# Autodesk Inventor assembly: Outer
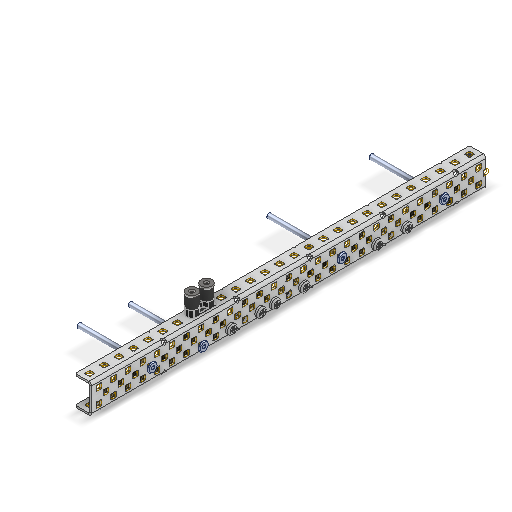
[picture p0: Inventor's stored thumbnail of the model, 512x512]
Saved by Autodesk Inventor 2025.2 (Build 292293000, 293)
## iProperties
Created: 2025-01-27
Part Number: Outer
Document SubType Name: Assembly
Designer: Averey Ku
Author: Averey Ku
## Documents named in this file (19)
- C:\Users\avere\VEX-CAD\V5-CAD\V0.2\Drivetrain\Drivebay Left\Outer.iam
- C:\Users\avere\VEX-CAD\ROBOPROS-CAD-Inventor\Motion\Shaft LS\Bearing Flat Low Profile.ipt
- C:\Users\avere\VEX-CAD\ROBOPROS-CAD-Inventor\Structure\Hardware\Screw Nylon - Pan Head\NScrew Pan Head Threaded .500.ipt
- C:\Users\avere\VEX-CAD\ROBOPROS-CAD-Inventor\Structure\Hardware\Screw Steel - Star\SScrew Star Smooth 2.500.ipt
- C:\Users\avere\VEX-CAD\ROBOPROS-CAD-Inventor\Structure\Hardware\Nut Keps.ipt
- C:\Users\avere\VEX-CAD\ROBOPROS-CAD-Inventor\Structure\Hardware\Nut Nylon\Nut Nylon - White.ipt
- C:\Users\avere\VEX-CAD\ROBOPROS-CAD-Inventor\Structure\C Channel\Aluminum 1x2x1\Alu C 1x2x1x28.ipt
- C:\Users\avere\VEX-CAD\ROBOPROS-CAD-Inventor\Structure\Standoff\Standoff .875.ipt
- C:\Users\avere\VEX-CAD\ROBOPROS-CAD-Inventor\Modified Parts\Bearing Flat Low Profile 2-Hole.ipt
- C:\Users\avere\VEX-CAD\ROBOPROS-CAD-Inventor\Motion\Spacers\Spacer Nylon .375 OD\NSpacer .375 OD x .375.ipt
- C:\Users\avere\VEX-CAD\ROBOPROS-CAD-Inventor\Motion\Spacers\Washer Steel\SWasher .375 OD x .062500.ipt
- C:\Users\avere\VEX-CAD\ROBOPROS-CAD-Inventor\Structure\Hardware\Screw Alu - Slotted\AScrew Slotted Threaded .250.ipt
- C:\Users\avere\VEX-CAD\ROBOPROS-CAD-Inventor\Structure\C Channel\Aluminum 1x2x1\Alu C 1x2x1x27.ipt
- C:\Users\avere\VEX-CAD\ROBOPROS-CAD-Inventor\Structure\Nylon Standoff Rounded\Nylon Standoff .875.ipt
- C:\Users\avere\VEX-CAD\ROBOPROS-CAD-Inventor\Structure\Hardware\Screw Steel - Star.ipt
- C:\Users\avere\VEX-CAD\ROBOPROS-CAD-Inventor\Structure\Hardware\Nut Nylon.ipt
- C:\Users\avere\VEX-CAD\ROBOPROS-CAD-Inventor\Structure\Standoff.ipt
- C:\Users\avere\VEX-CAD\ROBOPROS-CAD-Inventor\Motion\Spacers\Spacer Nylon .375 OD.ipt
- C:\Users\avere\VEX-CAD\ROBOPROS-CAD-Inventor\Motion\Spacers\Washer Steel.ipt
## Components (32 placed, 13 different names)
1. Bearing Flat Low Profile:2 — Insert:21, Insert:22, Insert:32, Mate:3
2. Bearing Flat Low Profile:3 — Insert:23, Insert:24, Insert:44
3. NScrew Pan Head Threaded .500:2 — Insert:35
4. NScrew Pan Head Threaded .500:3 — Insert:37
5. NScrew Pan Head Threaded .500:4 — Insert:36
6. NScrew Pan Head Threaded .500:5 — Insert:39, Mate:4
7. NScrew Pan Head Threaded .500:6 — Insert:38
8. SScrew Star Smooth 2.500:1 — Insert:27
9. SScrew Star Smooth 2.500:3 — Insert:26
10. SScrew Star Smooth 2.500:4 — Insert:25
11. Nut Keps:2 — Insert:43
12. Nut Keps:3 — Insert:41
13. Nut Keps:4 — Insert:42
14. Nut Nylon - White:2 — Insert:21
15. Nut Nylon - White:4 — Insert:22
16. Nut Nylon - White:5 — Insert:23, Mate:4
17. Nut Nylon - White:6 — Insert:24
18. Alu C 1x2x1x28:1 — Flush:1, Flush:2, Flush:3, Insert:25, Insert:26, Insert:27, Insert:31, Mate:2, Insert:32, Mate:3, Insert:35, Insert:36, Insert:37, Insert:38, Insert:39, Insert:40, Insert:41, Insert:42, Insert:43, Insert:44, Insert:45, Insert:46, Insert:48, Mate:5, Insert:53, Insert:54, Mate:6
19. Bearing Flat Low Profile:4 — Insert:31, Mate:2
20. Nut Nylon - White:7
21. Nut Nylon - White:8
22. NScrew Pan Head Threaded .500:8 — Insert:40
23. SScrew Star Smooth 2.500:5 — Insert:45
24. Standoff .875:1 — Insert:46
25. Bearing Flat Low Profile 2-Hole:1 — Insert:48, Mate:5, Insert:50, Insert:52
26. NSpacer .375 OD x .375:1 — Insert:49, Insert:50
27. SWasher .375 OD x .062500:1 — Insert:49
28. NSpacer .375 OD x .375:2 — Insert:52
29. SWasher .375 OD x .062500:2
30. AScrew Slotted Threaded .250:1 — Insert:53
31. Alu C 1x2x1x27:1 — Insert:54, Mate:6, Insert:55
32. Nylon Standoff .875:1 — Insert:55
## Relationships (39: Insert 31, Mate 5, Flush 3)
- Insert:21 (1.27 mm): Bearing Flat Low Profile:2 ↔ Nut Nylon - White:2
- Insert:22 (1.27 mm): Bearing Flat Low Profile:2 ↔ Nut Nylon - White:4
- Insert:23 (1.27 mm): Bearing Flat Low Profile:3 ↔ Nut Nylon - White:5
- Insert:24 (1.27 mm): Bearing Flat Low Profile:3 ↔ Nut Nylon - White:6
- Flush:1 (-177.8 mm): Alu C 1x2x1x28:1
- Flush:2 (-12.7 mm): Alu C 1x2x1x28:1
- Flush:3: Alu C 1x2x1x28:1
- Insert:25 (1.5875 mm): SScrew Star Smooth 2.500:4 ↔ Alu C 1x2x1x28:1
- Insert:26 (1.5875 mm): SScrew Star Smooth 2.500:3 ↔ Alu C 1x2x1x28:1
- Insert:27 (1.5875 mm): SScrew Star Smooth 2.500:1 ↔ Alu C 1x2x1x28:1
- [Insert] (1.27 mm): Bearing Flat Low Profile:4 ↔ Nut Nylon - White:7
- [Insert] (1.27 mm): Bearing Flat Low Profile:4 ↔ Nut Nylon - White:8
- Insert:31: Alu C 1x2x1x28:1 ↔ Bearing Flat Low Profile:4
- Mate:2: Alu C 1x2x1x28:1 ↔ Bearing Flat Low Profile:4
- Insert:32: Bearing Flat Low Profile:2 ↔ Alu C 1x2x1x28:1
- Mate:3: Bearing Flat Low Profile:2 ↔ Alu C 1x2x1x28:1
- Insert:35: NScrew Pan Head Threaded .500:2 ↔ Alu C 1x2x1x28:1
- Insert:36: NScrew Pan Head Threaded .500:4 ↔ Alu C 1x2x1x28:1
- Insert:37: NScrew Pan Head Threaded .500:3 ↔ Alu C 1x2x1x28:1
- Insert:38: NScrew Pan Head Threaded .500:6 ↔ Alu C 1x2x1x28:1
- Insert:39: NScrew Pan Head Threaded .500:5 ↔ Alu C 1x2x1x28:1
- Insert:40: Alu C 1x2x1x28:1 ↔ NScrew Pan Head Threaded .500:8
- Insert:41: Nut Keps:3 ↔ Alu C 1x2x1x28:1
- Insert:42: Nut Keps:4 ↔ Alu C 1x2x1x28:1
- Insert:43: Nut Keps:2 ↔ Alu C 1x2x1x28:1
- Insert:44: Bearing Flat Low Profile:3 ↔ Alu C 1x2x1x28:1
- Mate:4: NScrew Pan Head Threaded .500:5 ↔ Nut Nylon - White:5
- Insert:45 (1.5875 mm): Alu C 1x2x1x28:1 ↔ SScrew Star Smooth 2.500:5
- Insert:46: Alu C 1x2x1x28:1 ↔ Standoff .875:1
- Insert:48: Alu C 1x2x1x28:1 ↔ Bearing Flat Low Profile 2-Hole:1
- Mate:5: Alu C 1x2x1x28:1 ↔ Bearing Flat Low Profile 2-Hole:1
- Insert:49: NSpacer .375 OD x .375:1 ↔ SWasher .375 OD x .062500:1
- Insert:50 (1.27 mm): Bearing Flat Low Profile 2-Hole:1 ↔ NSpacer .375 OD x .375:1
- [Insert]: NSpacer .375 OD x .375:2 ↔ SWasher .375 OD x .062500:2
- Insert:52 (1.27 mm): Bearing Flat Low Profile 2-Hole:1 ↔ NSpacer .375 OD x .375:2
- Insert:53: Alu C 1x2x1x28:1 ↔ AScrew Slotted Threaded .250:1
- Insert:54: Alu C 1x2x1x28:1 ↔ Alu C 1x2x1x27:1
- Mate:6: Alu C 1x2x1x28:1 ↔ Alu C 1x2x1x27:1
- Insert:55: Alu C 1x2x1x27:1 ↔ Nylon Standoff .875:1
## Named parameters: d74_d57 = 1.27 mm, d75_d58 = 1.27 mm, d102_d100 = 0 mm
